# Autodesk Inventor assembly: KND-1000 Center 01
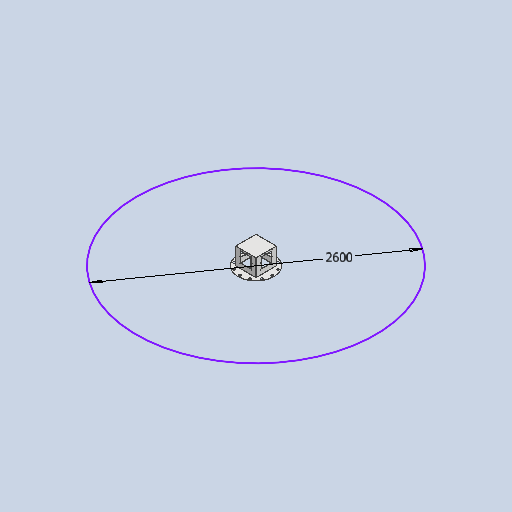
[picture p0: Inventor's stored thumbnail of the model, 512x512]
Saved by Autodesk Inventor 2026.2 (Build 302298000, 298)
## iProperties
Created: 2026-05-12
Part Number: KND-1000 Center 01
Document SubType Name: Assembly
Designer: admin
Stock Number: Центр
Author: admin
## Documents named in this file (4)
- C:\Users\admin\Documents\Inventor\KND-DistribSystem\DRS_D1200\KND-1000 Center 01.iam
- C:\Users\admin\Documents\Inventor\KND-DistribSystem\DRS_D1200\KND-9651 DrSysB MAIN FLANGE 01.ipt
- C:\Users\admin\Documents\Inventor\KND-DistribSystem\DRS_D1200\KND-1652 DrSysB Central tube wall 01.ipt
- C:\Users\admin\Documents\Inventor\KND-DistribSystem\DRS_D1200\KND-1665 DrSysB CUP 1 01.ipt
## Components (4 placed, 3 different names)
1. PRS 9651 DrSysB MAIN  FLANGE_D1200:1 — Flush:8, Flush:7, Mate:3
2. PRS 1652 DrSysB Central tube wall_D1200:1 — Flush:8, Flush:7, Mate:10, Rigid:22
3. PRS 1652 DrSysB Central tube wall_D1200:2 — Mate:3, Rigid:22
4. PRS 1665 DrSysB CUP 1_D1200:1 — Mate:10
## Relationships (5: Flush 2, Mate 2, WeldJoint 1)
- Flush:8: PRS 9651 DrSysB MAIN  FLANGE_D1200:1 ↔ PRS 1652 DrSysB Central tube wall_D1200:1
- Flush:7: PRS 9651 DrSysB MAIN  FLANGE_D1200:1 ↔ PRS 1652 DrSysB Central tube wall_D1200:1
- Mate:10: PRS 1652 DrSysB Central tube wall_D1200:1 ↔ PRS 1665 DrSysB CUP 1_D1200:1
- Mate:3: PRS 9651 DrSysB MAIN  FLANGE_D1200:1 ↔ PRS 1652 DrSysB Central tube wall_D1200:2
- Rigid:22 [WeldJoint]: PRS 1652 DrSysB Central tube wall_D1200:1 ↔ PRS 1652 DrSysB Central tube wall_D1200:2
